# Autodesk Inventor assembly: 39092
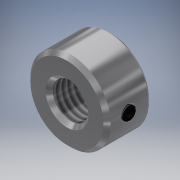
[picture p0: Inventor's stored thumbnail of the model, 180x180]
Saved by Autodesk Inventor 2019 (Build 230136000, 136)
## iProperties
Category: Collars
Company: Autodesk Inc.
Created: 2017-01-02
Part Number: 39092
Document SubType Name: Assembly
Designer: Autodesk Inc.
Catalog Web Link: http://www.tetrixrobotics.com/TETRIX_Axle_Set_Collars
Vendor: Tetrix
Author: Autodesk Inc.
## Documents named in this file (3)
- C:\Users\tbloo\Documents\Inventor\FTC Tetrix KOP\Tetrix_39092.iam
- C:\Users\tbloo\Downloads\FTC Tetrix KOP\Miscellaneous\Tetrix_39092_Collar.ipt
- C:\Users\tbloo\Downloads\FTC Tetrix KOP\Miscellaneous\Tetrix_39092_Screw.ipt
## Components (2 placed, 2 different names)
1. Tetrix_39092_Collar — Mate:1
2. Tetrix_39092_Screw — Mate:1
## Relationships (1: Mate 1)
- Mate:1: Tetrix_39092_Collar ↔ Tetrix_39092_Screw
